# Autodesk Inventor assembly: Assembly1
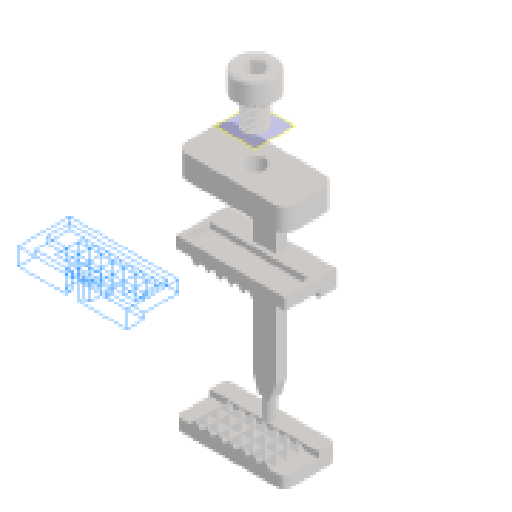
[picture p0: Inventor's stored thumbnail of the model, 512x512]
Saved by Autodesk Inventor 2023 (Build 270158000, 158)
## iProperties
Created: 2021-09-08
Part Number: Assembly1
Document SubType Name: Assembly
Designer: Nikita
Author: Nikita
## Documents named in this file (4)
- C:\Users\Public\GitHub-public\benchtop-hardware\Benchtop-2024(default-version)\custom-parts\sample_handling\Deprecated\Clamp-assembly.iam
- C:\Users\Public\GitHub-public\benchtop-hardware\Benchtop-2024(default-version)\custom-parts\sample_handling\Deprecated\gravity-clamp-base9x19mm-part1.ipt
- C:\Users\Public\GitHub-public\benchtop-hardware\Benchtop-2024(default-version)\custom-parts\sample_handling\Deprecated\gravity-clamp-base9x19mm-part2(moving).ipt
- C:\Users\Public\GitHub-public\benchtop-hardware\Benchtop-2024(default-version)\CAD-model-Inventor\library\Thorlabs\other\screwM4-12mm.ipt
## Components (3 placed, 3 different names)
1. gravity-clamp-base9x19mm-part1:1 — Mate:1, Mate:2, Mate:3
2. gravity-clamp-base9x19mm-part2(moving):3 — Mate:1, Mate:2, Mate:3
3. screwM4-12mm:1
## Relationships (3: Mate 3)
- Mate:1: gravity-clamp-base9x19mm-part1:1 ↔ gravity-clamp-base9x19mm-part2(moving):3
- Mate:2: gravity-clamp-base9x19mm-part1:1 ↔ gravity-clamp-base9x19mm-part2(moving):3
- Mate:3: gravity-clamp-base9x19mm-part1:1 ↔ gravity-clamp-base9x19mm-part2(moving):3
